# Autodesk Inventor assembly: Female_Tail_v2
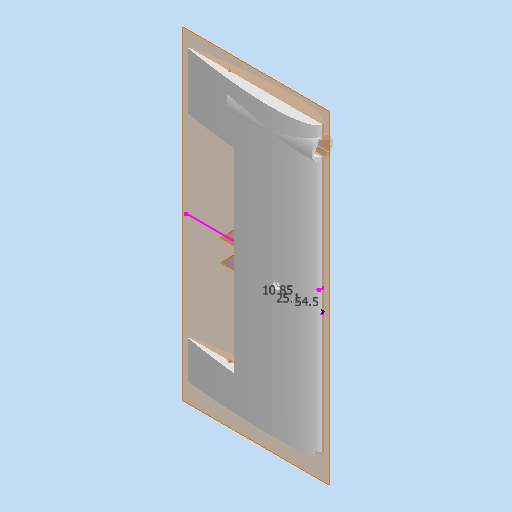
[picture p0: Inventor's stored thumbnail of the model, 512x512]
Saved by Autodesk Inventor 2027 (Build 310192060, 192F)
## iProperties
Created: 2026-08-06
Part Number: Female_Tail_v2
Document SubType Name: Assembly
Designer: Delbe
Author: Delbe
## Documents named in this file (3)
- C:\GitHub\SWIFT-UAV\System_development\Pelican\structural_model\v0.3.0\Parts\Delb_Parts\Old_Models_and_Mich\Female_Tail_v2.iam
- C:\GitHub\SWIFT-UAV\System_development\Pelican\structural_model\v0.3.0\Parts\Delb_Parts\Female_Tail_Female_Connector.ipt
- C:\GitHub\SWIFT-UAV\System_development\Pelican\structural_model\v0.3.0\Parts\Delb_Parts\Female_Tail_Male_Connector.ipt
## Components (2 placed, 2 different names)
1. Female_Tail_Female_Connector:1 — Rigid:1
2. Female_Tail_Male_Connector:1 — Rigid:1
## Relationships (1: WeldJoint 1)
- Rigid:1 [WeldJoint]: Female_Tail_Female_Connector:1 ↔ Female_Tail_Male_Connector:1
